# Autodesk Inventor assembly: BancEcoShell
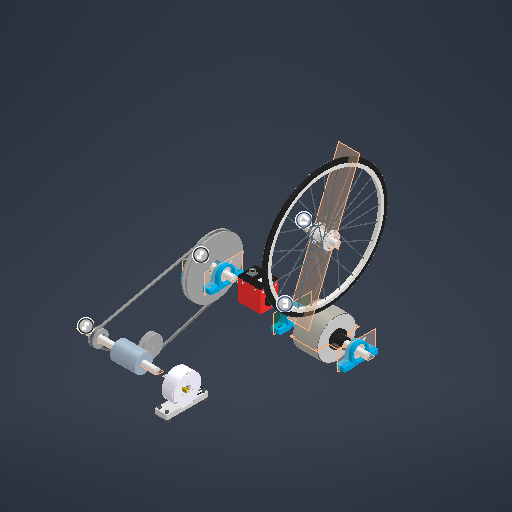
[picture p0: Inventor's stored thumbnail of the model, 512x512]
Saved by Autodesk Inventor 2026.2 (Build 302298010, 298A)
## iProperties
Created: 2026-03-31
Part Number: BancEcoShell
Document SubType Name: Assembly
Designer: romai
Author: romai
## Documents named in this file (17)
- D:\Downloads\LogicielMaster\Inventor\Enssemble\BancEcoShell\BancEcoShell.iam
- D:\Downloads\LogicielMaster\Inventor\Pièces\Couplemètre.ipt
- D:\Downloads\LogicielMaster\Inventor\Pièces\Rouleau.ipt
- C:\Users\romai\Documents\Inventor\Content Center Files\R2026\fr-FR\ISO 1207(2)\ISO 1207 - M2 x 3.ipt
- D:\Downloads\LogicielMaster\Inventor\Enssemble\BancEcoShell\ArbreRoue1.ipt
- D:\Downloads\LogicielMaster\Inventor\Enssemble\BancEcoShell\ArbreCouplemètre1.ipt
- D:\Downloads\LogicielMaster\Inventor\Pièces\RoueVelo.ipt
- D:\Downloads\LogicielMaster\Inventor\Enssemble\BancEcoShell\ArbrePrimaire2.ipt
- D:\Downloads\LogicielMaster\Inventor\Enssemble\BancEcoShell\ArbreRoue2.ipt
- D:\Downloads\LogicielMaster\Inventor\Enssemble\BancEcoShell\ArbreSecondaire2.ipt
- D:\Downloads\LogicielMaster\Inventor\Enssemble\BancEcoShell\BancEcoShell\Design Accelerator\Transmission par courroie trapézoïdale2.iam
- D:\Downloads\LogicielMaster\Inventor\Pièces\Frein.ipt
- D:\Downloads\LogicielMaster\Inventor\Enssemble\BancEcoShell\ArbrePoulie1.ipt
- D:\Downloads\LogicielMaster\Inventor\Enssemble\BancEcoShell\SupportArbre.ipt
- D:\Downloads\LogicielMaster\Inventor\Enssemble\BancEcoShell\Palier.ipt
- D:\Downloads\LogicielMaster\Inventor\Enssemble\BancEcoShell\Flasque.ipt
- D:\Downloads\LogicielMaster\Inventor\Enssemble\BancEcoShell\Masse.ipt
## Components (24 placed, 16 different names)
1. Couplemètre:1 — Placage:1, Placage:2, Placage:3, Affleurement:5, Placage:10, Placage:11, Placage:15, Placage:16
2. ArbreCouplemètre:1 — Placage:3, Affleurement:5, Placage:5, Placage:6, Angle:1, Placage:13, Placage:14, Angle:4
3. ArbrePrimaire:2 — Placage:5, Placage:6, Placage:7, Placage:8, Angle:1, Angle:2, Placage:24, Placage:25, Placage:28, Placage:29, Placage:34, Placage:35
4. Rouleau:1 — Placage:7, Placage:8, Angle:2, Rotation:1, Placage:9, Placage:26, Placage:27, Angle:8, Angle:9
5. RoueVelo:1 — Rotation:1, Placage:9, Placage:10, Placage:11, Placage:12, Affleurement:1, Angle:3
6. ArbreRoue:1 — Placage:12, Affleurement:1, Angle:3
7. ArbreSecondaire:1 — Affleurement:2, Placage:15, Placage:16, Placage:17, Affleurement:3, Angle:6, Angle:7, Placage:22, Placage:23, Placage:40, Angle:17
8. ArbrePoulie:1 — Placage:13, Placage:14, Angle:4, Affleurement:2, Placage:18, Angle:5, Placage:30, Placage:38
9. Transmission par courroie trapézoïdale:1 [sub-assembly] — Placage:17, Placage:18, Affleurement:3, Angle:5, Angle:6, Placage:33, Placage:39, Placage:41
10. Frein:1 — Placage:19, Placage:20, Placage:21, Placage:22, Angle:16
11. ArbreFrein:1 — Placage:19, Placage:20, Placage:21, Angle:7, Placage:23
12. SupportArbre:1 — Placage:24, Placage:26, Angle:8, Placage:31, Placage:36, Angle:10
13. SupportArbre:2 — Placage:25, Placage:27, Angle:9, Placage:32, Placage:37, Angle:11
14. Palier:1 — Placage:28, Placage:31, Angle:12
15. Palier:2 — Placage:29, Placage:32, Angle:13
16. Palier:3 — Placage:30, Placage:33, Angle:14
17. Flasque:1 — Placage:34, Placage:36, Angle:10
18. Flasque:2 — Placage:35, Placage:37, Angle:11
19. Palier:4 — Placage:38, Placage:39, Angle:15
20. Masse:1 — Placage:40, Placage:41, Angle:17
21. ISO 1207 M2 x 3:1 — Placage:1, Placage:2
22. ISO 1207 M2 x 3:2
23. ISO 1207 M2 x 3:3
24. ISO 1207 M2 x 3:4
## Component patterns: (4 elements, first: ISO 1207 M2 x 3:1)
## Relationships (62: Mate 40, Angle 17, Flush 4, RelateRotation 1)
- Placage:1 [Mate]: Couplemètre:1 ↔ ISO 1207 M2 x 3:1
- Placage:2 [Mate]: Couplemètre:1 ↔ ISO 1207 M2 x 3:1
- Placage:3 [Mate]: Couplemètre:1 ↔ ArbreCouplemètre:1
- Affleurement:5 [Flush]: Couplemètre:1 ↔ ArbreCouplemètre:1
- Placage:5 [Mate]: ArbreCouplemètre:1 ↔ ArbrePrimaire:2
- Placage:6 [Mate] (23.6 mm): ArbreCouplemètre:1 ↔ ArbrePrimaire:2
- Placage:7 [Mate]: ArbrePrimaire:2 ↔ Rouleau:1
- Placage:8 [Mate]: ArbrePrimaire:2 ↔ Rouleau:1
- Angle:1 (0 deg): ArbreCouplemètre:1 ↔ ArbrePrimaire:2
- Angle:2 (0 deg): ArbrePrimaire:2 ↔ Rouleau:1
- Rotation:1 [RelateRotation] (8.25 ul): Rouleau:1 ↔ RoueVelo:1
- Placage:9 [Mate]: Rouleau:1 ↔ RoueVelo:1
- Placage:10 [Mate]: Couplemètre:1 ↔ RoueVelo:1
- Placage:11 [Mate] (278 mm): Couplemètre:1 ↔ RoueVelo:1
- Placage:12 [Mate]: RoueVelo:1 ↔ ArbreRoue:1
- Affleurement:1 [Flush] (-25 mm): RoueVelo:1 ↔ ArbreRoue:1
- Angle:3 (0 deg): RoueVelo:1 ↔ ArbreRoue:1
- Placage:13 [Mate] (23.6 mm): ArbreCouplemètre:1 ↔ ArbrePoulie:1
- Placage:14 [Mate]: ArbreCouplemètre:1 ↔ ArbrePoulie:1
- Angle:4 (0 deg): ArbreCouplemètre:1 ↔ ArbrePoulie:1
- Affleurement:2 [Flush]: ArbreSecondaire:1 ↔ ArbrePoulie:1
- Placage:15 [Mate] (467 mm): Couplemètre:1 ↔ ArbreSecondaire:1
- Placage:16 [Mate] (-75 mm): Couplemètre:1 ↔ ArbreSecondaire:1
- Placage:17 [Mate]: ArbreSecondaire:1 ↔ Transmission par courroie trapézoïdale:1
- Placage:18 [Mate]: ArbrePoulie:1 ↔ Transmission par courroie trapézoïdale:1
- Affleurement:3 [Flush] (50 mm): ArbreSecondaire:1 ↔ Transmission par courroie trapézoïdale:1
- Angle:5 (0 deg): ArbrePoulie:1 ↔ Transmission par courroie trapézoïdale:1
- Angle:6 (0 deg): ArbreSecondaire:1 ↔ Transmission par courroie trapézoïdale:1
- Placage:19 [Mate]: Frein:1 ↔ ArbreFrein:1
- Placage:20 [Mate]: Frein:1 ↔ ArbreFrein:1
- Placage:21 [Mate]: Frein:1 ↔ ArbreFrein:1
- Angle:7 (0 deg): ArbreSecondaire:1 ↔ ArbreFrein:1
- Placage:22 [Mate]: ArbreSecondaire:1 ↔ Frein:1
- Placage:23 [Mate] (35 mm): ArbreSecondaire:1 ↔ ArbreFrein:1
- Placage:24 [Mate]: ArbrePrimaire:2 ↔ SupportArbre:1
- Placage:25 [Mate]: ArbrePrimaire:2 ↔ SupportArbre:2
- Placage:26 [Mate]: Rouleau:1 ↔ SupportArbre:1
- Placage:27 [Mate]: Rouleau:1 ↔ SupportArbre:2
- Angle:8 (0 deg): Rouleau:1 ↔ SupportArbre:1
- Angle:9 (0 deg): Rouleau:1 ↔ SupportArbre:2
- Placage:28 [Mate]: ArbrePrimaire:2 ↔ Palier:1
- Placage:29 [Mate]: ArbrePrimaire:2 ↔ Palier:2
- Placage:30 [Mate]: ArbrePoulie:1 ↔ Palier:3
- Placage:31 [Mate] (20 mm): SupportArbre:1 ↔ Palier:1
- Placage:32 [Mate] (20 mm): SupportArbre:2 ↔ Palier:2
- Placage:33 [Mate] (10 mm): Transmission par courroie trapézoïdale:1 ↔ Palier:3
- Placage:34 [Mate]: ArbrePrimaire:2 ↔ Flasque:1
- Placage:35 [Mate]: ArbrePrimaire:2 ↔ Flasque:2
- Placage:36 [Mate]: SupportArbre:1 ↔ Flasque:1
- Placage:37 [Mate]: SupportArbre:2 ↔ Flasque:2
- Angle:10 (0 deg): SupportArbre:1 ↔ Flasque:1
- Angle:11 (0 deg): SupportArbre:2 ↔ Flasque:2
- Angle:12 (180 deg): Palier:1
- Angle:13 (180 deg): Palier:2
- Angle:14 (180 deg): Palier:3
- Placage:38 [Mate]: ArbrePoulie:1 ↔ Palier:4
- Placage:39 [Mate] (10 mm): Transmission par courroie trapézoïdale:1 ↔ Palier:4
- Angle:15 (180 deg): Palier:4
- Angle:16 (180 deg): Frein:1
- Placage:40 [Mate]: ArbreSecondaire:1 ↔ Masse:1
- Placage:41 [Mate] (75 mm): Transmission par courroie trapézoïdale:1 ↔ Masse:1
- Angle:17 (0 deg): ArbreSecondaire:1 ↔ Masse:1
